# Autodesk Inventor assembly: Assembly
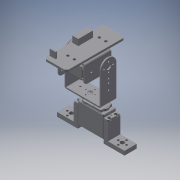
[picture p0: Inventor's stored thumbnail of the model, 180x180]
Saved by Autodesk Inventor 2016 (Build 200138000, 138)
## iProperties
Created: 2016-01-27
Part Number: Assembly
Document SubType Name: Assembly
Designer: seve
Author: seve
## Documents named in this file (6)
- C:\Users\seve\ccup\CAD\dual-servo\Assembly.iam
- C:\Users\seve\ccup\CAD\dual-servo\ext\hitec-hs-325hb-1.snapshot.1\Hitec HS-325HB.iam
- C:\Users\seve\ccup\CAD\dual-servo\ext\hitec-hs-325hb-1.snapshot.1\Multi Purpose Bracket.ipt
- C:\Users\seve\ccup\CAD\dual-servo\ext\hitec-hs-325hb-1.snapshot.1\U Long Bracket.ipt
- C:\Users\seve\ccup\CAD\dual-servo\LaserMount.ipt
- C:\Users\seve\ccup\CAD\dual-servo\base_bracket.ipt
## Components (7 placed, 5 different names)
1. Hitec HS-325HB:1 [sub-assembly] — Insert:1, Angle:1, Flush:2, Mate:1, Insert:4
2. Hitec HS-325HB:2 [sub-assembly] — Insert:2, Insert:3, Angle:2
3. U Long Bracket:1 — Insert:1, Angle:1, Insert:2
4. Multi Purpose Bracket:2 — Insert:3, Angle:2, Flush:1, Angle:4, Insert:5
5. LaserMount:1 — Flush:1, Angle:3, Angle:4, Insert:5
6. base_bracket:1 — Flush:2, Angle:3
7. base_bracket:2 — Mate:1, Insert:4
## Relationships (12: Insert 5, Angle 4, Flush 2, Mate 1)
- Insert:1: Hitec HS-325HB:1 ↔ U Long Bracket:1
- Angle:1 (0 deg): Hitec HS-325HB:1 ↔ U Long Bracket:1
- Insert:2: Hitec HS-325HB:2 ↔ U Long Bracket:1
- Insert:3: Hitec HS-325HB:2 ↔ Multi Purpose Bracket:2
- Angle:2 (180 deg): Hitec HS-325HB:2 ↔ Multi Purpose Bracket:2
- Flush:1: Multi Purpose Bracket:2 ↔ LaserMount:1
- Flush:2: Hitec HS-325HB:1 ↔ base_bracket:1
- Mate:1: Hitec HS-325HB:1 ↔ base_bracket:2
- Insert:4: Hitec HS-325HB:1 ↔ base_bracket:2
- Angle:3 (0 deg): LaserMount:1 ↔ base_bracket:1
- Angle:4 (0 deg): Multi Purpose Bracket:2 ↔ LaserMount:1
- Insert:5: Multi Purpose Bracket:2 ↔ LaserMount:1
